# Autodesk Inventor assembly: AERO - Assembly
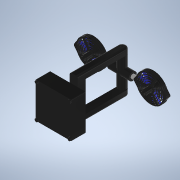
[picture p0: Inventor's stored thumbnail of the model, 180x180]
Saved by Autodesk Inventor 2021 (Build 250183000, 183)
## iProperties
Created: 2021-01-21
Part Number: AERO - Assembly
Document SubType Name: Assembly
Designer: garciar1
Author: garciar1
## Documents named in this file (6)
- C:\Users\garciar1\Dropbox\Tutoring\MCEN90017_Motion Control\2021\Assignments\Resources\Models\AERO Digital Twin\AERO - Assembly.iam
- C:\Users\garciar1\Dropbox\Tutoring\MCEN90017_Motion Control\2021\Assignments\Resources\Models\AERO Digital Twin\Components\AERO - Base.ipt
- C:\Users\garciar1\Dropbox\Tutoring\MCEN90017_Motion Control\2021\Assignments\Resources\Models\AERO Digital Twin\Components\AERO - Fork.ipt
- C:\Users\garciar1\Dropbox\Tutoring\MCEN90017_Motion Control\2021\Assignments\Resources\Models\AERO Digital Twin\Components\AERO - Arm.ipt
- C:\Users\garciar1\Dropbox\Tutoring\MCEN90017_Motion Control\2021\Assignments\Resources\Models\AERO Digital Twin\Components\AERO - Propeller Housing.ipt
- C:\Users\garciar1\Dropbox\Tutoring\MCEN90017_Motion Control\2021\Assignments\Resources\Models\AERO Digital Twin\Components\AERO - Propeller.ipt
## Components (7 placed, 5 different names)
1. AERO - Base:1 — Rotational:1
2. AERO - Fork:1 — Rotational:1, Rotational:2
3. AERO - Arm:1 — Rotational:2, Rotational:3, Rotational:4
4. AERO - Propeller Housing:1 — Rotational:3, Rotational:5
5. AERO - Propeller Housing:2 — Rotational:4, Rotational:6
6. AERO - Propeller:1 — Rotational:5
7. AERO - Propeller:2 — Rotational:6
## Relationships (6: RevoluteJoint 6)
- Rotational:1 [RevoluteJoint]: AERO - Base:1 ↔ AERO - Fork:1
- Rotational:2 [RevoluteJoint]: AERO - Fork:1 ↔ AERO - Arm:1
- Rotational:3 [RevoluteJoint]: AERO - Arm:1 ↔ AERO - Propeller Housing:1
- Rotational:4 [RevoluteJoint]: AERO - Arm:1 ↔ AERO - Propeller Housing:2
- Rotational:5 [RevoluteJoint]: AERO - Propeller Housing:1 ↔ AERO - Propeller:1
- Rotational:6 [RevoluteJoint]: AERO - Propeller Housing:2 ↔ AERO - Propeller:2
